# Autodesk Inventor assembly: PlanetaryGear
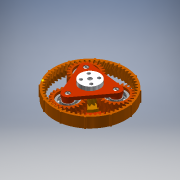
[picture p0: Inventor's stored thumbnail of the model, 180x180]
Saved by Autodesk Inventor 2018.3 (Build 223284000, 284)
## iProperties
Created: 2018-07-08
Part Number: PlanetaryGear
Material: Generisch
Document SubType Name: Assembly
Designer: JochenAlt
Author: JochenAlt
## Documents named in this file (11)
- D:\Projects\FlowerPot\CAD\PlanetaryGear\PlanetaryGear.iam
- D:\Projects\FlowerPot\CAD\PlanetaryGear\Konstruktions-Assistent\Stirnzahnrad21.ipt
- D:\Projects\FlowerPot\CAD\PlanetaryGear\Konstruktions-Assistent\Stirnzahnrad23.ipt
- D:\Projects\FlowerPot\CAD\PlanetaryGear\PlanetaryHolder.ipt
- D:\Projects\FlowerPot\CAD\PlanetaryGear\PlanetaryHolderTop.ipt
- D:\Projects\FlowerPot\CAD\Mounting Hub.ipt
- D:\Projects\FlowerPot\CAD\PlanetaryGear\PlanetaryHolderBottom.ipt
- D:\Projects\FlowerPot\CAD\PlanetaryGear\PlanetaryGearConstr\Konstruktions-Assistent\Stirnzahnrad12.ipt
- C:\Users\JochenAlt\Documents\Inventor\Content Center Files\R2018\de-DE\DIN BEARING(1)\DIN 625 SKF - SKF 626.ipt
- C:\Users\JochenAlt\Documents\Inventor\Content Center Files\R2018\de-DE\DIN 912\DIN 912 - M2 x 0,4 x 12 x 11.ipt
- C:\Users\JochenAlt\Documents\Inventor\Content Center Files\R2018\de-DE\DIN 934\DIN 934 - M2 x 0,4.ipt
## Components (18 placed, 9 different names)
1. Stirnzahnrad2:1 — Fluchtend:1, Fluchtend:2, Fluchtend:3, Passend:57, Passend:66, Fluchtend:7
2. Stirnzahnrad2:2 — Fluchtend:2, Passend:46, Fluchtend:4, Drehung:3
3. Stirnzahnrad2:3 — Fluchtend:1, Fluchtend:6, Passend:47, Drehung:2
4. Stirnzahnrad2:4 — Passend:34, Fluchtend:3, Fluchtend:5, Drehung:4
5. PlanetaryHolder:1
6. PlanetaryHolderTop:1 — Passend:48, Passend:49, Passend:50, Passend:51, Passend:52, Passend:53, Passend:54, Passend:55, Passend:56, Passend:57, Passend:58, Passend:59, Drehung:5
7. Mounting Hub:1 — Passend:58, Passend:59, Drehung:5
8. PlanetaryHolderBottom:1 — Passend:60, Passend:61, Passend:62, Passend:63, Passend:64, Passend:65, Drehung:1, Drehung:2, Drehung:3, Drehung:4
9. Stirnzahnrad1:1 — Passend:66, Fluchtend:7, Drehung:1
10. DIN 625 SKF SKF 626:1 — Passend:46, Fluchtend:4, Passend:48, Passend:60
11. DIN 625 SKF SKF 626:2 — Passend:34, Fluchtend:5, Passend:50, Passend:51
12. DIN 625 SKF SKF 626:3 — Fluchtend:6, Passend:47, Passend:49
13. DIN 912 - ersetzt durch DIN EN ISO 4762 M2 x 12:1 — Passend:45, Passend:56, Passend:65
14. DIN 912 - ersetzt durch DIN EN ISO 4762 M2 x 12:2 — Passend:43, Passend:54, Passend:63, Passend:64
15. DIN 912 - ersetzt durch DIN EN ISO 4762 M2 x 12:3 — Passend:41, Passend:52, Passend:61, Passend:62
16. DIN 934 - ersetzt durch DIN EN 24032/28673/28674 M2:1 — Passend:41, Passend:53
17. DIN 934 - ersetzt durch DIN EN 24032/28673/28674 M2:2 — Passend:43, Passend:55
18. DIN 934 - ersetzt durch DIN EN 24032/28673/28674 M2:3 — Passend:45
## Relationships (37: Mate 25, Flush 7, RelateRotation 5)
- Passend:34 [Mate]: Stirnzahnrad2:4 ↔ DIN 625 SKF SKF 626:2
- Passend:41 [Mate]: DIN 912 - ersetzt durch DIN EN ISO 4762 M2 x 12:3 ↔ DIN 934 - ersetzt durch DIN EN 24032/28673/28674 M2:1
- Passend:43 [Mate]: DIN 912 - ersetzt durch DIN EN ISO 4762 M2 x 12:2 ↔ DIN 934 - ersetzt durch DIN EN 24032/28673/28674 M2:2
- Passend:45 [Mate]: DIN 912 - ersetzt durch DIN EN ISO 4762 M2 x 12:1 ↔ DIN 934 - ersetzt durch DIN EN 24032/28673/28674 M2:3
- Fluchtend:1 [Flush]: Stirnzahnrad2:1 ↔ Stirnzahnrad2:3
- Fluchtend:2 [Flush]: Stirnzahnrad2:1 ↔ Stirnzahnrad2:2
- Fluchtend:3 [Flush]: Stirnzahnrad2:1 ↔ Stirnzahnrad2:4
- Passend:46 [Mate]: Stirnzahnrad2:2 ↔ DIN 625 SKF SKF 626:1
- Fluchtend:4 [Flush] (2 mm): Stirnzahnrad2:2 ↔ DIN 625 SKF SKF 626:1
- Fluchtend:5 [Flush] (2 mm): Stirnzahnrad2:4 ↔ DIN 625 SKF SKF 626:2
- Fluchtend:6 [Flush] (2 mm): Stirnzahnrad2:3 ↔ DIN 625 SKF SKF 626:3
- Passend:47 [Mate]: Stirnzahnrad2:3 ↔ DIN 625 SKF SKF 626:3
- Passend:48 [Mate]: PlanetaryHolderTop:1 ↔ DIN 625 SKF SKF 626:1
- Passend:49 [Mate]: PlanetaryHolderTop:1 ↔ DIN 625 SKF SKF 626:3
- Passend:50 [Mate]: PlanetaryHolderTop:1 ↔ DIN 625 SKF SKF 626:2
- Passend:51 [Mate]: PlanetaryHolderTop:1 ↔ DIN 625 SKF SKF 626:2
- Passend:52 [Mate]: PlanetaryHolderTop:1 ↔ DIN 912 - ersetzt durch DIN EN ISO 4762 M2 x 12:3
- Passend:53 [Mate]: PlanetaryHolderTop:1 ↔ DIN 934 - ersetzt durch DIN EN 24032/28673/28674 M2:1
- Passend:54 [Mate]: PlanetaryHolderTop:1 ↔ DIN 912 - ersetzt durch DIN EN ISO 4762 M2 x 12:2
- Passend:55 [Mate]: PlanetaryHolderTop:1 ↔ DIN 934 - ersetzt durch DIN EN 24032/28673/28674 M2:2
- Passend:56 [Mate]: PlanetaryHolderTop:1 ↔ DIN 912 - ersetzt durch DIN EN ISO 4762 M2 x 12:1
- Passend:57 [Mate]: Stirnzahnrad2:1 ↔ PlanetaryHolderTop:1
- Passend:58 [Mate]: PlanetaryHolderTop:1 ↔ Mounting Hub:1
- Passend:59 [Mate]: PlanetaryHolderTop:1 ↔ Mounting Hub:1
- Passend:60 [Mate]: PlanetaryHolderBottom:1 ↔ DIN 625 SKF SKF 626:1
- Passend:61 [Mate]: PlanetaryHolderBottom:1 ↔ DIN 912 - ersetzt durch DIN EN ISO 4762 M2 x 12:3
- Passend:62 [Mate]: PlanetaryHolderBottom:1 ↔ DIN 912 - ersetzt durch DIN EN ISO 4762 M2 x 12:3
- Passend:63 [Mate]: PlanetaryHolderBottom:1 ↔ DIN 912 - ersetzt durch DIN EN ISO 4762 M2 x 12:2
- Passend:64 [Mate]: PlanetaryHolderBottom:1 ↔ DIN 912 - ersetzt durch DIN EN ISO 4762 M2 x 12:2
- Passend:65 [Mate]: PlanetaryHolderBottom:1 ↔ DIN 912 - ersetzt durch DIN EN ISO 4762 M2 x 12:1
- Passend:66 [Mate]: Stirnzahnrad2:1 ↔ Stirnzahnrad1:1
- Fluchtend:7 [Flush]: Stirnzahnrad2:1 ↔ Stirnzahnrad1:1
- Drehung:1 [RelateRotation] (-0.2 ul): PlanetaryHolderBottom:1 ↔ Stirnzahnrad1:1
- Drehung:2 [RelateRotation] (1.5 ul): Stirnzahnrad2:3 ↔ PlanetaryHolderBottom:1
- Drehung:3 [RelateRotation] (1.5 ul): Stirnzahnrad2:2 ↔ PlanetaryHolderBottom:1
- Drehung:4 [RelateRotation] (1.5 ul): Stirnzahnrad2:4 ↔ PlanetaryHolderBottom:1
- Drehung:5 [RelateRotation] (1 ul): PlanetaryHolderTop:1 ↔ Mounting Hub:1
